# Autodesk Inventor assembly: Head_
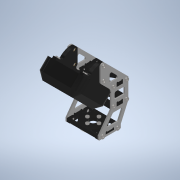
[picture p0: Inventor's stored thumbnail of the model, 180x180]
Saved by Autodesk Inventor 2020.4 (Build 244396000, 396)
## iProperties
Created: 2021-12-31
Part Number: Head_
Document SubType Name: Assembly
Designer: Masato Kubotera
Mass: 94.5268 g
Surface Area: 553.647 cm^2
Volume: 95.1642 cm^3
Density: 0.993302 g/cm^3
Author: Masato Kubotera
## Documents named in this file (12)
- C:\Users\Masato\Documents\Inventor\CIT Brains_Inventor\OpenPlatform_ver3_0 - ve4_1 branch\UpperBody\Head\Head_.iam
- C:\Users\Masato\Documents\Inventor\CIT Brains_Inventor\OpenPlatform_ver3_0 - ve4_1 branch\UpperBody\Head\CameraUnit.iam
- C:\Users\Masato\Documents\Inventor\CIT Brains_Inventor\OpenPlatform_ver3_0 - ve4_1 branch\UpperBody\Head\Camera_side_frame_.ipt
- C:\Users\Masato\Documents\Inventor\CIT Brains_Inventor\OpenPlatform_ver3_0 - ve4_1 branch\Ready_Made\UD-43040.ipt
- C:\Users\Masato\Documents\Inventor\CIT Brains_Inventor\OpenPlatform_ver3_0 - ve4_1 branch\Ready_Made\Screw\M3-10.ipt
- C:\Users\Masato\Documents\Inventor\CIT Brains_Inventor\OpenPlatform_ver3_0 - ve4_1 branch\UpperBody\Head\Head_side_frame_.ipt
- C:\Users\Masato\Documents\Inventor\CIT Brains_Inventor\OpenPlatform_ver3_0 - ve4_1 branch\Ready_Made\Screw\M3-6.ipt
- C:\Users\Masato\Documents\Inventor\CIT Brains_Inventor\OpenPlatform_ver3_0 - ve4_1 branch\UpperBody\Head\Head_horn_frame_.ipt
- C:\Users\Masato\Documents\Inventor\CIT Brains_Inventor\OpenPlatform_ver3_0 - ve4_1 branch\Ready_Made\IRU-304SW.ipt
- C:\Users\Masato\Documents\Inventor\CIT Brains_Inventor\OpenPlatform_ver3_0 - ve4_1 branch\Ready_Made\TT-2532-10.ipt
- C:\Users\Masato\Documents\Inventor\CIT Brains_Inventor\OpenPlatform_ver3_0 - ve4_1 branch\Ready_Made\Screw\M2_6-8.ipt
- C:\Users\Masato\Documents\Inventor\CIT Brains_Inventor\OpenPlatform_ver3_0 - ve4_1 branch\UpperBody\Head\Head_diagonal_.ipt
## Components (49 placed, 11 different names)
1. CameraUnit:1 [sub-assembly] — 挿入:1, 挿入:2, 挿入:3, 挿入:4
2. Camera_side_frame_:1 — 挿入:1, 挿入:2, 挿入:5, 挿入:6, 挿入:9, 挿入:10
3. Camera_side_frame_:2 — 挿入:3, 挿入:4, 挿入:7, 挿入:8, 挿入:11, 挿入:12
4. UD-43040:1 — 挿入:5, 挿入:13
5. UD-43040:2 — 挿入:6, 挿入:14
6. UD-43040:3 — 挿入:7, 挿入:15
7. UD-43040:4 — 挿入:8, 挿入:16
8. M3-10:1 — 挿入:9
9. M3-10:2 — 挿入:10
10. M3-10:3 — 挿入:11
11. M3-10:4 — 挿入:12
12. Head_side_frame_:1 — 挿入:13, 挿入:14, 挿入:17, 挿入:18, 挿入:25, 挿入:26, 挿入:34, 挿入:35, 挿入:46, 挿入:47, 挿入:52, 挿入:53, 挿入:54, 挿入:55, 挿入:58, 挿入:59
13. Head_side_frame_:2 — 挿入:15, 挿入:16, 挿入:19, 挿入:20, 挿入:27, 挿入:28, 挿入:36, 挿入:37, 挿入:48, 挿入:49, 挿入:50, 挿入:51, 挿入:56, 挿入:57, 挿入:60, 挿入:61
14. M3-6:1 — 挿入:17
15. M3-6:2 — 挿入:18
16. M3-6:3 — 挿入:19
17. M3-6:4 — 挿入:20
18. Head_horn_frame_:1 — 挿入:21, 挿入:22, 挿入:23, 挿入:24, 挿入:29, 挿入:30, 挿入:31, 挿入:32, 挿入:33, メイト:1, メイト:2, メイト:3
19. IRU-304SW:1 — 挿入:21, 挿入:25
20. IRU-304SW:2 — 挿入:22, 挿入:26
21. IRU-304SW:3 — 挿入:23, 挿入:28
22. IRU-304SW:4 — 挿入:24, 挿入:27
23. TT-2532-10:1 — 挿入:29
24. M2_6-8:1 — 挿入:30
25. M2_6-8:2 — 挿入:31
26. M2_6-8:3 — 挿入:32
27. M2_6-8:4 — 挿入:33
28. M3-6:5 — 挿入:34
29. M3-6:6 — 挿入:35
30. M3-6:7 — 挿入:36
31. M3-6:8 — 挿入:37
32. Head_diagonal_:1 — 挿入:38, 挿入:39, 挿入:40, 挿入:41
33. Head_diagonal_:2 — 挿入:42, 挿入:43, 挿入:44, 挿入:45
34. IRU-304SW:5 — 挿入:38, 挿入:46
35. IRU-304SW:6 — 挿入:39, 挿入:47
36. IRU-304SW:7 — 挿入:40, 挿入:48
37. IRU-304SW:8 — 挿入:41, 挿入:49
38. IRU-304SW:9 — 挿入:42, 挿入:53
39. IRU-304SW:10 — 挿入:43, 挿入:52
40. IRU-304SW:11 — 挿入:44, 挿入:50
41. IRU-304SW:12 — 挿入:45, 挿入:51
42. M3-6:9 — 挿入:54
43. M3-6:10 — 挿入:55
44. M3-6:11 — 挿入:56
45. M3-6:12 — 挿入:57
46. M3-6:13 — 挿入:58
47. M3-6:14 — 挿入:59
48. M3-6:15 — 挿入:60
49. M3-6:16 — 挿入:61
## Relationships (64: Insert 61, Mate 3)
- 挿入:1 [Insert]: CameraUnit:1 ↔ Camera_side_frame_:1
- 挿入:2 [Insert]: CameraUnit:1 ↔ Camera_side_frame_:1
- 挿入:3 [Insert]: CameraUnit:1 ↔ Camera_side_frame_:2
- 挿入:4 [Insert]: CameraUnit:1 ↔ Camera_side_frame_:2
- 挿入:5 [Insert]: Camera_side_frame_:1 ↔ UD-43040:1
- 挿入:6 [Insert]: Camera_side_frame_:1 ↔ UD-43040:2
- 挿入:7 [Insert]: Camera_side_frame_:2 ↔ UD-43040:3
- 挿入:8 [Insert]: Camera_side_frame_:2 ↔ UD-43040:4
- 挿入:9 [Insert]: Camera_side_frame_:1 ↔ M3-10:1
- 挿入:10 [Insert]: Camera_side_frame_:1 ↔ M3-10:2
- 挿入:11 [Insert]: Camera_side_frame_:2 ↔ M3-10:3
- 挿入:12 [Insert]: Camera_side_frame_:2 ↔ M3-10:4
- 挿入:13 [Insert]: UD-43040:1 ↔ Head_side_frame_:1
- 挿入:14 [Insert]: UD-43040:2 ↔ Head_side_frame_:1
- 挿入:15 [Insert]: UD-43040:3 ↔ Head_side_frame_:2
- 挿入:16 [Insert]: UD-43040:4 ↔ Head_side_frame_:2
- 挿入:17 [Insert]: Head_side_frame_:1 ↔ M3-6:1
- 挿入:18 [Insert]: Head_side_frame_:1 ↔ M3-6:2
- 挿入:19 [Insert]: Head_side_frame_:2 ↔ M3-6:3
- 挿入:20 [Insert]: Head_side_frame_:2 ↔ M3-6:4
- 挿入:21 [Insert]: Head_horn_frame_:1 ↔ IRU-304SW:1
- 挿入:22 [Insert]: Head_horn_frame_:1 ↔ IRU-304SW:2
- 挿入:23 [Insert]: Head_horn_frame_:1 ↔ IRU-304SW:3
- 挿入:24 [Insert]: Head_horn_frame_:1 ↔ IRU-304SW:4
- 挿入:25 [Insert]: Head_side_frame_:1 ↔ IRU-304SW:1
- 挿入:26 [Insert]: Head_side_frame_:1 ↔ IRU-304SW:2
- 挿入:27 [Insert]: Head_side_frame_:2 ↔ IRU-304SW:4
- 挿入:28 [Insert]: Head_side_frame_:2 ↔ IRU-304SW:3
- 挿入:29 [Insert]: Head_horn_frame_:1 ↔ TT-2532-10:1
- 挿入:30 [Insert]: Head_horn_frame_:1 ↔ M2_6-8:1
- 挿入:31 [Insert]: Head_horn_frame_:1 ↔ M2_6-8:2
- 挿入:32 [Insert]: Head_horn_frame_:1 ↔ M2_6-8:3
- 挿入:33 [Insert]: Head_horn_frame_:1 ↔ M2_6-8:4
- 挿入:34 [Insert]: Head_side_frame_:1 ↔ M3-6:5
- 挿入:35 [Insert]: Head_side_frame_:1 ↔ M3-6:6
- 挿入:36 [Insert]: Head_side_frame_:2 ↔ M3-6:7
- 挿入:37 [Insert]: Head_side_frame_:2 ↔ M3-6:8
- 挿入:38 [Insert]: Head_diagonal_:1 ↔ IRU-304SW:5
- 挿入:39 [Insert]: Head_diagonal_:1 ↔ IRU-304SW:6
- 挿入:40 [Insert]: Head_diagonal_:1 ↔ IRU-304SW:7
- 挿入:41 [Insert]: Head_diagonal_:1 ↔ IRU-304SW:8
- 挿入:42 [Insert]: Head_diagonal_:2 ↔ IRU-304SW:9
- 挿入:43 [Insert]: Head_diagonal_:2 ↔ IRU-304SW:10
- 挿入:44 [Insert]: Head_diagonal_:2 ↔ IRU-304SW:11
- 挿入:45 [Insert]: Head_diagonal_:2 ↔ IRU-304SW:12
- 挿入:46 [Insert]: Head_side_frame_:1 ↔ IRU-304SW:5
- 挿入:47 [Insert]: Head_side_frame_:1 ↔ IRU-304SW:6
- 挿入:48 [Insert]: Head_side_frame_:2 ↔ IRU-304SW:7
- 挿入:49 [Insert]: Head_side_frame_:2 ↔ IRU-304SW:8
- 挿入:50 [Insert]: Head_side_frame_:2 ↔ IRU-304SW:11
- 挿入:51 [Insert]: Head_side_frame_:2 ↔ IRU-304SW:12
- 挿入:52 [Insert]: Head_side_frame_:1 ↔ IRU-304SW:10
- 挿入:53 [Insert]: Head_side_frame_:1 ↔ IRU-304SW:9
- 挿入:54 [Insert]: Head_side_frame_:1 ↔ M3-6:9
- 挿入:55 [Insert]: Head_side_frame_:1 ↔ M3-6:10
- 挿入:56 [Insert]: Head_side_frame_:2 ↔ M3-6:11
- 挿入:57 [Insert]: Head_side_frame_:2 ↔ M3-6:12
- 挿入:58 [Insert]: Head_side_frame_:1 ↔ M3-6:13
- 挿入:59 [Insert]: Head_side_frame_:1 ↔ M3-6:14
- 挿入:60 [Insert]: Head_side_frame_:2 ↔ M3-6:15
- 挿入:61 [Insert]: Head_side_frame_:2 ↔ M3-6:16
- メイト:1 [Mate]: Head_horn_frame_:1
- メイト:2 [Mate]: Head_horn_frame_:1
- メイト:3 [Mate]: Head_horn_frame_:1
